# Autodesk Inventor assembly: Pendulum Suspension Assembly
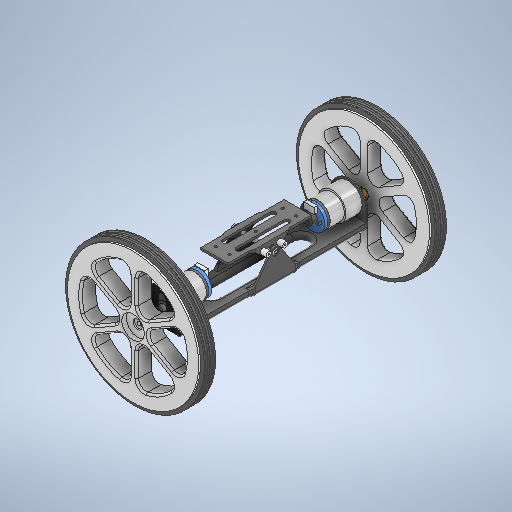
[picture p0: Inventor's stored thumbnail of the model, 512x512]
Saved by Autodesk Inventor 2025.2 (Build 292293000, 293)
## iProperties
Created: 2025-01-23
Part Number: Pendulum Suspension Assembly
Document SubType Name: Assembly
Designer: Matt Tidd
Author: Matt Tidd
## Documents named in this file (11)
- C:\Users\mtidd2\Desktop\H2A\CAD\Motors_and_Wheels\Pendulum Suspension\Pendulum Suspension Assembly.iam
- C:\Users\mtidd2\Desktop\H2A\CAD\Motors_and_Wheels\Pendulum Suspension\Pendulum Bottom Bracket.ipt
- C:\Users\mtidd2\Desktop\H2A\CAD\Motors_and_Wheels\Pendulum Suspension\Rotation Pin.ipt
- C:\Users\mtidd2\Desktop\H2A\CAD\Motors_and_Wheels\Pendulum Suspension\Rotation Bearing.ipt
- C:\Users\mtidd2\Desktop\H2A\CAD\Motors_and_Wheels\Pendulum Suspension\Rotation End Cap.ipt
- C:\Users\mtidd2\Desktop\H2A\CAD\Motors_and_Wheels\Pendulum Suspension\Pendulum Top Bracket.ipt
- C:\Users\mtidd2\Desktop\H2A\CAD\Motors_and_Wheels\520 DC Gear Motor.ipt
- C:\Users\mtidd2\Desktop\H2A\CAD\Motors_and_Wheels\Pendulum Suspension\Rotation Bumper.ipt
- C:\Users\mtidd2\Desktop\H2A\CAD\Motors_and_Wheels\Wheel Assembly\520 DC Gear Motor Wheel Coupler.ipt
- C:\Users\mtidd2\Desktop\H2A\CAD\Motors_and_Wheels\Wheel Assembly\PLA Wheel Frame.ipt
- C:\Users\mtidd2\Desktop\H2A\CAD\Motors_and_Wheels\Wheel Assembly\TPU Tire.ipt
## Components (17 placed, 10 different names)
1. Pendulum Bottom Bracket:1 — Rotational:1, Rotational:6, Mate:1, Mate:2, Mate:3, Mate:4, Mate:5, Mate:6, Pendulum Rotational Joint
2. Rotation Pin:1 — Rotational:2
3. Rotation Bearing:1 — Rotational:3, Rotational:4
4. Rotation End Cap:1 — Rotational:6
5. Rotation Bearing:2 — Rotational:5
6. Rotation End Cap:2 — Rotational:1, Rotational:2, Rotational:3
7. Pendulum Top Bracket:1 — Rotational:4, Rotational:5, Rigid:1, Rigid:2, Pendulum Rotational Joint
8. 520 DC Gear Motor:1 — Mate:1, Mate:2, Mate:3, Rotational:8
9. 520 DC Gear Motor:2 — Mate:4, Mate:5, Mate:6, Rotational:7
10. Rotation Bumper:1 — Rigid:1
11. Rotation Bumper:2 — Rigid:2
12. 520 DC Gear Motor Wheel Coupler:1 — Rotational:8, Rotational:9
13. 520 DC Gear Motor Wheel Coupler:2 — Rotational:7, Rigid:3
14. PLA Wheel Frame:1 — Rotational:9, Mate:8, Mate:9
15. PLA Wheel Frame:2 — Rigid:3, Mate:7, Mate:10
16. TPU Tire:1 — Mate:8, Mate:9
17. TPU Tire:2 — Mate:7, Mate:10
## Relationships (23: RevoluteJoint 10, Mate 10, WeldJoint 3)
- Rotational:1 [RevoluteJoint]: Pendulum Bottom Bracket:1 ↔ Rotation End Cap:2
- Rotational:2 [RevoluteJoint]: Rotation Pin:1 ↔ Rotation End Cap:2
- Rotational:3 [RevoluteJoint]: Rotation Bearing:1 ↔ Rotation End Cap:2
- Rotational:4 [RevoluteJoint]: Rotation Bearing:1 ↔ Pendulum Top Bracket:1
- Rotational:5 [RevoluteJoint]: Rotation Bearing:2 ↔ Pendulum Top Bracket:1
- Rotational:6 [RevoluteJoint]: Pendulum Bottom Bracket:1 ↔ Rotation End Cap:1
- Rigid:1 [WeldJoint]: Pendulum Top Bracket:1 ↔ Rotation Bumper:1
- Rigid:2 [WeldJoint]: Pendulum Top Bracket:1 ↔ Rotation Bumper:2
- Mate:1: Pendulum Bottom Bracket:1 ↔ 520 DC Gear Motor:1
- Mate:2: Pendulum Bottom Bracket:1 ↔ 520 DC Gear Motor:1
- Mate:3: Pendulum Bottom Bracket:1 ↔ 520 DC Gear Motor:1
- Mate:4: Pendulum Bottom Bracket:1 ↔ 520 DC Gear Motor:2
- Mate:5: Pendulum Bottom Bracket:1 ↔ 520 DC Gear Motor:2
- Mate:6: Pendulum Bottom Bracket:1 ↔ 520 DC Gear Motor:2
- Rotational:7 [RevoluteJoint]: 520 DC Gear Motor:2 ↔ 520 DC Gear Motor Wheel Coupler:2
- Rotational:8 [RevoluteJoint]: 520 DC Gear Motor:1 ↔ 520 DC Gear Motor Wheel Coupler:1
- Rigid:3 [WeldJoint]: 520 DC Gear Motor Wheel Coupler:2 ↔ PLA Wheel Frame:2
- Mate:7: PLA Wheel Frame:2 ↔ TPU Tire:2
- Rotational:9 [RevoluteJoint]: 520 DC Gear Motor Wheel Coupler:1 ↔ PLA Wheel Frame:1
- Mate:8: PLA Wheel Frame:1 ↔ TPU Tire:1
- Mate:9: PLA Wheel Frame:1 ↔ TPU Tire:1
- Mate:10: PLA Wheel Frame:2 ↔ TPU Tire:2
- Pendulum Rotational Joint [RevoluteJoint] (6 mm): Pendulum Bottom Bracket:1 ↔ Pendulum Top Bracket:1
